# Autodesk Inventor assembly: Rulment
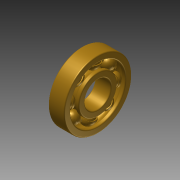
[picture p0: Inventor's stored thumbnail of the model, 180x180]
Saved by Autodesk Inventor 2011 SP2 (Build 150309200, 309)
## iProperties
Created: 2023-03-13
Part Number: Rulment
Document SubType Name: Assembly
Designer: utilizator
Author: utilizator
## Documents named in this file (5)
- D:\Studenti\Donisan Enya 1322b\Lab 3 - Rulment\Rulment.iam
- D:\Studenti\Donisan Enya 1322b\Lab 3 - Rulment\InelExterior.ipt
- D:\Studenti\Donisan Enya 1322b\Lab 3 - Rulment\InelInterior.ipt
- D:\Studenti\Donisan Enya 1322b\Lab 3 - Rulment\Bila.ipt
- D:\Studenti\Donisan Enya 1322b\Lab 3 - Rulment\Curea.ipt
## Components (12 placed, 4 different names)
1. InelExterior:1 — Mate:1, Mate:2, Mate:3, Tangent:1
2. InelInterior:1 — Mate:1, Mate:2, Mate:4, Mate:5, Mate:6, Mate:7
3. Curea:1 — Mate:5, Mate:6, Mate:7, Insert:1, Insert:2
4. Curea:2 — Insert:1, Insert:2
5. Bila:1 — Mate:3, Tangent:1, Mate:4
6. Bila:2
7. Bila:3
8. Bila:4
9. Bila:5
10. Bila:6
11. Bila:7
12. Bila:8
## Component patterns: (8 elements, first: Bila:1)
## Relationships (10: Mate 7, Insert 2, Tangent 1)
- Mate:1: InelExterior:1 ↔ InelInterior:1
- Mate:2: InelExterior:1 ↔ InelInterior:1
- Mate:3: InelExterior:1 ↔ Bila:1
- Tangent:1: InelExterior:1 ↔ Bila:1
- Mate:4: InelInterior:1 ↔ Bila:1
- Mate:5: InelInterior:1 ↔ Curea:1
- Mate:6: InelInterior:1 ↔ Curea:1
- Mate:7: InelInterior:1 ↔ Curea:1
- Insert:1: Curea:1 ↔ Curea:2
- Insert:2: Curea:1 ↔ Curea:2
